# Autodesk Inventor assembly: Desk
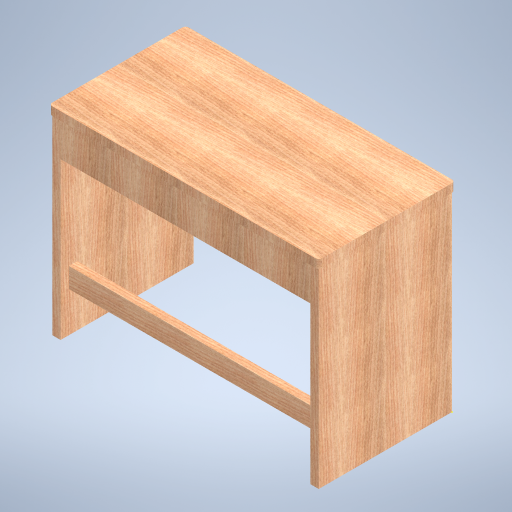
[picture p0: Inventor's stored thumbnail of the model, 512x512]
Saved by Autodesk Inventor 2023 (Build 270158000, 158)
## iProperties
Created: 2022-09-18
Part Number: Desk
Document SubType Name: Assembly
Designer: mliu-23
Author: mliu-23
## Documents named in this file (3)
- D:\MyProfile\Documents\GitHub\VirtualPeddie\CommonObj\CommonObj_Universal\(Desk)CommonObj_Universal_Desk\Desk.iam
- D:\MyProfile\Documents\GitHub\VirtualPeddie\CommonObj\CommonObj_Universal\(Desk)CommonObj_Universal_Desk\Desk.ipt
- D:\MyProfile\Documents\GitHub\VirtualPeddie\CommonObj\CommonObj_Universal\(Desk)CommonObj_Universal_Desk\Drawer.ipt
## Components (2 placed, 2 different names)
1. Desk:1 — Mate:1, Flush:1
2. Drawer:1 — Mate:1, Flush:1
## Relationships (2: Mate 1, Flush 1)
- Mate:1: Desk:1 ↔ Drawer:1
- Flush:1: Desk:1 ↔ Drawer:1
